# Autodesk Inventor assembly: YMotorassembly
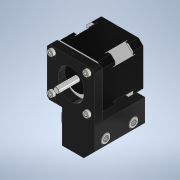
[picture p0: Inventor's stored thumbnail of the model, 180x180]
Saved by Autodesk Inventor 2020.2 (Build 242310000, 310)
## iProperties
Created: 2020-08-25
Part Number: YMotorassembly
Document SubType Name: Assembly
Designer: JK
Author: JK
## Documents named in this file (6)
- C:\Users\JK\Documents\Inventor\Anet Upgrade\YMotorassembly.iam
- C:\Users\JK\Documents\Inventor\Anet Upgrade\ymotorholder.ipt
- C:\Users\JK\Documents\Inventor\Anet Upgrade\MOTOR.ipt
- C:\Users\JK\Documents\Inventor\Anet Upgrade\M3x10.ipt
- C:\Users\JK\Documents\Inventor\Anet Upgrade\M5x30Bolt.ipt
- C:\Users\JK\Documents\Inventor\Anet Upgrade\T_Slot_Nut_Dropin_3030m5ipt.ipt
## Components (10 placed, 5 different names)
1. ymotorholder:1 — Mate:1, Angle:1, Mate:2, Mate:7, Mate:8, Mate:9, Mate:10, Angle:2, Mate:13
2. MOTOR:1 — Mate:1, Angle:1, Mate:2, Mate:3, Mate:4, Mate:5, Mate:6
3. M3x10:1 — Mate:4, Flush:2
4. M3x10:2 — Mate:3, Flush:1, Flush:2
5. M3x10:3 — Mate:5, Flush:3
6. M3x10:4 — Mate:6, Flush:1, Flush:3, Mate:7
7. M5x30Bolt:1 — Mate:9, Mate:10, Flush:4, Mate:11
8. M5x30Bolt:2 — Mate:8, Flush:4, Mate:12
9. T_Slot_Nut_Dropin_3030m5ipt:1 — Mate:11, Angle:2, Angle:3, Flush:5, Mate:13
10. T_Slot_Nut_Dropin_3030m5ipt:2 — Mate:12, Angle:3, Flush:5
## Relationships (21: Mate 13, Flush 5, Angle 3)
- Mate:1: ymotorholder:1 ↔ MOTOR:1
- Angle:1 (0 deg): ymotorholder:1 ↔ MOTOR:1
- Mate:2: ymotorholder:1 ↔ MOTOR:1
- Mate:3: MOTOR:1 ↔ M3x10:2
- Mate:4: MOTOR:1 ↔ M3x10:1
- Mate:5: MOTOR:1 ↔ M3x10:3
- Mate:6: MOTOR:1 ↔ M3x10:4
- Flush:1: M3x10:2 ↔ M3x10:4
- Flush:2: M3x10:1 ↔ M3x10:2
- Flush:3: M3x10:3 ↔ M3x10:4
- Mate:7: ymotorholder:1 ↔ M3x10:4
- Mate:8: ymotorholder:1 ↔ M5x30Bolt:2
- Mate:9: ymotorholder:1 ↔ M5x30Bolt:1
- Mate:10: ymotorholder:1 ↔ M5x30Bolt:1
- Flush:4: M5x30Bolt:1 ↔ M5x30Bolt:2
- Mate:11: M5x30Bolt:1 ↔ T_Slot_Nut_Dropin_3030m5ipt:1
- Mate:12: M5x30Bolt:2 ↔ T_Slot_Nut_Dropin_3030m5ipt:2
- Angle:2 (0 deg): ymotorholder:1 ↔ T_Slot_Nut_Dropin_3030m5ipt:1
- Angle:3 (0 deg): T_Slot_Nut_Dropin_3030m5ipt:1 ↔ T_Slot_Nut_Dropin_3030m5ipt:2
- Flush:5: T_Slot_Nut_Dropin_3030m5ipt:1 ↔ T_Slot_Nut_Dropin_3030m5ipt:2
- Mate:13: ymotorholder:1 ↔ T_Slot_Nut_Dropin_3030m5ipt:1
